# Autodesk Inventor assembly: ArmSolenoid
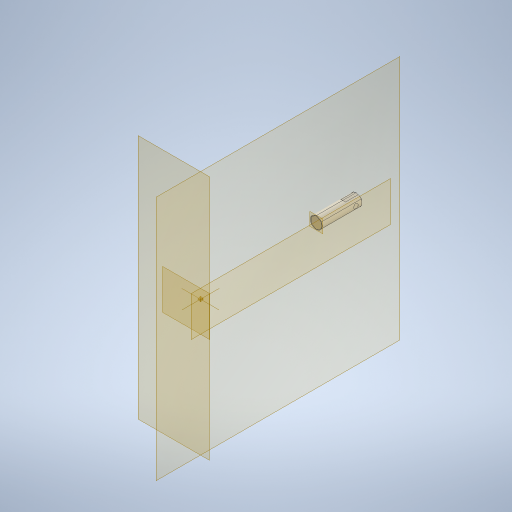
[picture p0: Inventor's stored thumbnail of the model, 512x512]
Saved by Autodesk Inventor 2023 (Build 270158000, 158)
## iProperties
Created: 2023-03-29
Part Number: ArmSolenoid
Document SubType Name: Assembly
Designer: LattePanda
Author: LattePanda
## Documents named in this file (6)
- C:\Users\LattePanda\Desktop\str1ker\parts\external\ArmSolenoid.iam
- C:\Users\LattePanda\Desktop\str1ker\parts\external\ArmSolenoidBody.ipt
- C:\Users\LattePanda\Desktop\str1ker\parts\SolenoidBracket.ipt
- C:\Users\LattePanda\Desktop\str1ker\parts\external\ArmSolenoidShaft.ipt
- C:\Users\LattePanda\Desktop\str1ker\description\models\src\ArmSolenoidBoundingBoc.ipt
- C:\Users\LattePanda\Desktop\str1ker\description\models\ArmSolenoidShaftBoundingBox.ipt
## Components (5 placed, 5 different names)
1. ArmSolenoid:1 — Mate:4, Mate:9, Angle:1, Mate:10, Mate:11
2. SolenoidBracket:1 — Mate:4, Mate:7, Mate:8, Mate:9, Flush:5
3. ArmSolenoidShaft:1 — Mate:10, Angle:2, Mate:11, Flush:9
4. ArmSolenoidBoundingBoc:1 — Flush:1, Flush:2, Mate:12, Flush:5
5. ArmSolenoidShaftBoundingBox:1 — Flush:6, Flush:7, Flush:8, Mate:13, Flush:9
## Relationships (17: Mate 8, Flush 7, Angle 2)
- Mate:4: ArmSolenoid:1 ↔ SolenoidBracket:1
- Mate:7: SolenoidBracket:1
- Mate:8: SolenoidBracket:1
- Mate:9: ArmSolenoid:1 ↔ SolenoidBracket:1
- Angle:1 (0 deg): ArmSolenoid:1
- Mate:10: ArmSolenoid:1 ↔ ArmSolenoidShaft:1
- Angle:2 (0 deg): ArmSolenoidShaft:1
- Mate:11 (6 mm): ArmSolenoid:1 ↔ ArmSolenoidShaft:1
- Flush:1: ArmSolenoidBoundingBoc:1
- Flush:2: ArmSolenoidBoundingBoc:1
- Mate:12: ArmSolenoidBoundingBoc:1
- Flush:5: SolenoidBracket:1 ↔ ArmSolenoidBoundingBoc:1
- Flush:6: ArmSolenoidShaftBoundingBox:1
- Flush:7: ArmSolenoidShaftBoundingBox:1
- Flush:8: ArmSolenoidShaftBoundingBox:1
- Mate:13: ArmSolenoidShaftBoundingBox:1
- Flush:9: ArmSolenoidShaft:1 ↔ ArmSolenoidShaftBoundingBox:1
